# Autodesk Inventor assembly: thigh_right
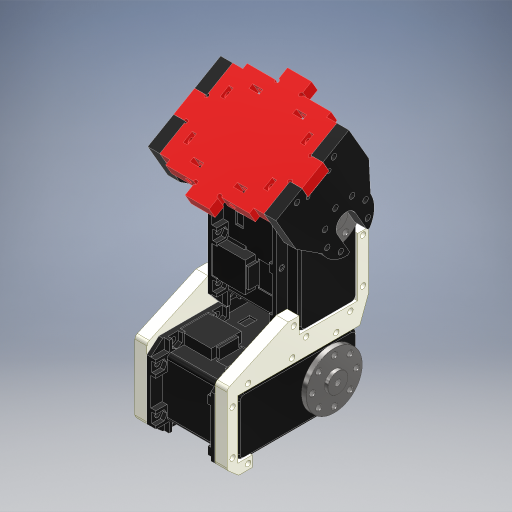
[picture p0: Inventor's stored thumbnail of the model, 512x512]
Saved by Autodesk Inventor 2024 (Build 280153000, 153)
## iProperties
Created: 2024-09-15
Part Number: thigh_right
Document SubType Name: Assembly
Designer: msi
Author: msi
## Documents named in this file (7)
- C:\Users\msi\GITHUB\19th_intern_kgh_fight_robot\부품\Lower_Body\Thigh\thigh_left.iam
- C:\Users\msi\GITHUB\19th_intern_kgh_fight_robot\부품\Lower_Body\Thigh\64_106 fixation.ipt
- C:\Users\msi\GITHUB\19th_intern_kgh_fight_robot\부품\Lower_Body\Thigh\knee fixation.ipt
- C:\Users\msi\GITHUB\19th_intern_kgh_fight_robot\부품\Lower_Body\Thigh\hip joint and thigh connection_106.ipt
- C:\Users\msi\GITHUB\19th_intern_kgh_fight_robot\부품\ROBOTIS(Inventor 2024 ver.)\다이나믹셀\MX-106T+idle.ipt.iam
- C:\Users\msi\GITHUB\19th_intern_kgh_fight_robot\부품\ROBOTIS(Inventor 2024 ver.)\혼\64-106Horn.ipt
- MX-106T+idle.ipt
## Components (9 placed, 5 different names)
1. knee fixation:1 — 삽입:1, 삽입:2, 삽입:17, 삽입:18
2. hip joint and thigh connection_106:1 — 삽입:6, 삽입:7, 삽입:9, 삽입:10
3. MX-106T+idle.ipt:1 [sub-assembly] — 삽입:1, 삽입:2, 삽입:3, 삽입:4, 삽입:5, 삽입:8
4. MX-106T+idle.ipt:2 [sub-assembly] — 삽입:17, 삽입:18, 삽입:19, 삽입:20, 삽입:21
5. 64-106Horn:1 — 삽입:5, 삽입:6, 삽입:7
6. 64_106 fixation:1 — 삽입:9, 삽입:10, 삽입:11, 삽입:12
7. knee fixation:2 — 삽입:3, 삽입:4, 삽입:19, 삽입:20
8. hip joint and thigh connection_106:2 — 삽입:8, 삽입:11, 삽입:12
9. 64-106Horn:2 — 삽입:21
## Relationships (17: Insert 17)
- 삽입:1 [Insert]: knee fixation:1 ↔ MX-106T+idle.ipt:1
- 삽입:2 [Insert]: knee fixation:1 ↔ MX-106T+idle.ipt:1
- 삽입:3 [Insert]: MX-106T+idle.ipt:1 ↔ knee fixation:2
- 삽입:4 [Insert]: MX-106T+idle.ipt:1 ↔ knee fixation:2
- 삽입:5 [Insert]: MX-106T+idle.ipt:1 ↔ 64-106Horn:1
- 삽입:6 [Insert]: hip joint and thigh connection_106:1 ↔ 64-106Horn:1
- 삽입:7 [Insert]: hip joint and thigh connection_106:1 ↔ 64-106Horn:1
- 삽입:8 [Insert]: MX-106T+idle.ipt:1 ↔ hip joint and thigh connection_106:2
- 삽입:9 [Insert]: hip joint and thigh connection_106:1 ↔ 64_106 fixation:1
- 삽입:10 [Insert]: hip joint and thigh connection_106:1 ↔ 64_106 fixation:1
- 삽입:11 [Insert]: 64_106 fixation:1 ↔ hip joint and thigh connection_106:2
- 삽입:12 [Insert]: 64_106 fixation:1 ↔ hip joint and thigh connection_106:2
- 삽입:17 [Insert]: knee fixation:1 ↔ MX-106T+idle.ipt:2
- 삽입:18 [Insert]: knee fixation:1 ↔ MX-106T+idle.ipt:2
- 삽입:19 [Insert]: MX-106T+idle.ipt:2 ↔ knee fixation:2
- 삽입:20 [Insert]: MX-106T+idle.ipt:2 ↔ knee fixation:2
- 삽입:21 [Insert]: MX-106T+idle.ipt:2 ↔ 64-106Horn:2
